# Autodesk Inventor assembly: Cut Profile
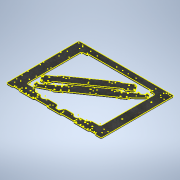
[picture p0: Inventor's stored thumbnail of the model, 180x180]
Saved by Autodesk Inventor 2020 (Build 240168000, 168)
## iProperties
Created: 2019-10-11
Part Number: Cut Profile
Document SubType Name: Assembly
Designer: pepd9
Author: pepd9
## Documents named in this file (5)
- C:\DESIGNS\MK3PRO P1\FRAME\Cut Profile.iam
- C:\DESIGNS\MK3PRO P1\FRAME\FRONT PLATE P1.2.ipt
- C:\DESIGNS\MK3PRO P1\FRAME\REAR PLATE P1.2.ipt
- C:\DESIGNS\MK3PRO P1\FRAME\CENTER FRAME P1.2.ipt
- C:\DESIGNS\MK3PRO P1\FRAME\CUT SKETCH.ipt
## Components (4 placed, 4 different names)
1. FRONT PLATE P1.2:1 — Flush:2, Angle:2
2. REAR PLATE P1.2:1 — Flush:1, Angle:1
3. CENTER FRAME P1.2:1 — Flush:1, Flush:2, Angle:1, Angle:2, Flush:3, Flush:4
4. CUT SKETCH:1 — Flush:3, Flush:4
## Relationships (6: Flush 4, Angle 2)
- Flush:1: REAR PLATE P1.2:1 ↔ CENTER FRAME P1.2:1
- Flush:2: FRONT PLATE P1.2:1 ↔ CENTER FRAME P1.2:1
- Angle:1 (145 deg): REAR PLATE P1.2:1 ↔ CENTER FRAME P1.2:1
- Angle:2 (145 deg): FRONT PLATE P1.2:1 ↔ CENTER FRAME P1.2:1
- Flush:3: CENTER FRAME P1.2:1 ↔ CUT SKETCH:1
- Flush:4: CENTER FRAME P1.2:1 ↔ CUT SKETCH:1
